# Autodesk Inventor assembly: LGA 771 Passive Heatsink
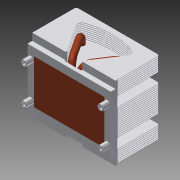
[picture p0: Inventor's stored thumbnail of the model, 180x180]
Saved by Autodesk Inventor 2015 (Build 190159000, 159)
## iProperties
Created: 2015-08-21
Part Number: LGA 771 Passive Heatsink
Document SubType Name: Assembly
Designer: Kyle
Author: Kyle
## Documents named in this file (7)
- C:\Users\Kyle\Documents\Project documentation\Supermicro X7DCA-L Watercooling\LGA 771 Passive Heatsink.iam
- C:\Users\Kyle\Documents\Project documentation\Supermicro X7DCA-L Watercooling\Heatsink_base_al.ipt
- C:\Users\Kyle\Documents\Project documentation\Supermicro X7DCA-L Watercooling\Heatsink_base_cu.ipt
- C:\Users\Kyle\Documents\Project documentation\Supermicro X7DCA-L Watercooling\Fin_full.ipt
- C:\Users\Kyle\Documents\Project documentation\Supermicro X7DCA-L Watercooling\Fin_short.ipt
- C:\Users\Kyle\Documents\Project documentation\Supermicro X7DCA-L Watercooling\Fin_holed.ipt
- C:\Users\Kyle\Documents\Project documentation\Supermicro X7DCA-L Watercooling\Heatpipe.iam
## Components (47 placed, 6 different names)
1. Heatsink_base_al:1 — Mate:1, Mate:2, Flush:1, Mate:7, Flush:2, Flush:3, Mate:8, Flush:4, Mate:10, Flush:5, Mate:12, Flush:6, Mate:14, Flush:7, Mate:16, Flush:8, Mate:18, Flush:9, Mate:20, Flush:10, Mate:22, Flush:11, Mate:24, Mate:26, Mate:28, Mate:30, Mate:32, Flush:16, Mate:34, Flush:17, Mate:36, Flush:18, Mate:38, Flush:19, Mate:40, Flush:20, Mate:42, Flush:21, Mate:44, Flush:22, Mate:46, Flush:23, Mate:48, Flush:24, Mate:50, Flush:25, Mate:52, Flush:26, Mate:54, Flush:27, Mate:56, Flush:28, Mate:58, Flush:29, Mate:60, Flush:30, Mate:62, Flush:31, Mate:64, Mate:66, Mate:68, Mate:70, Mate:72, Mate:74, Flush:37, Mate:76, Flush:38, Mate:78, Flush:39, Mate:80, Flush:40, Mate:82, Flush:41, Mate:84, Flush:42, Mate:86, Flush:43, Mate:88, Flush:44, Mate:90, Flush:45
2. Heatsink_base_cu:1 — Mate:1, Mate:2, Flush:1, Mate:92, Mate:93, Mate:94, Mate:95
3. Fin_full:1 — Mate:7, Flush:2, Flush:3, Mate:9, Tangent:1, Tangent:2, Tangent:3
4. Fin_full:2 — Mate:20, Flush:10, Mate:21, Mate:23
5. Fin_full:3 — Mate:18, Flush:9, Mate:19, Mate:21
6. Fin_full:4 — Mate:16, Flush:8, Mate:17, Mate:19
7. Fin_full:5 — Mate:12, Flush:6, Mate:13, Mate:15
8. Fin_full:6 — Mate:10, Flush:5, Mate:11, Mate:13
9. Fin_full:7 — Mate:8, Flush:4, Mate:9, Mate:11
10. Fin_full:8 — Mate:14, Flush:7, Mate:15, Mate:17
11. Fin_short:1 — Mate:30, Flush:15, Mate:31, Mate:33, Flush:32
12. Fin_short:2 — Mate:28, Mate:29, Flush:14, Flush:15, Mate:31
13. Fin_short:3 — Mate:26, Flush:13, Mate:27, Mate:29, Flush:14
14. Fin_short:4 — Mate:24, Flush:12, Mate:25, Flush:13, Mate:27
15. Fin_short:5 — Mate:22, Flush:11, Mate:23, Flush:12, Mate:25
16. Fin_full:9 — Mate:62, Flush:31, Mate:63, Mate:65
17. Fin_full:10 — Mate:60, Flush:30, Mate:61, Mate:63
18. Fin_full:11 — Mate:58, Flush:29, Mate:59, Mate:61
19. Fin_full:12 — Mate:56, Flush:28, Mate:57, Mate:59
20. Fin_full:13 — Mate:54, Flush:27, Mate:55, Mate:57
21. Fin_full:14 — Mate:52, Flush:26, Mate:53, Mate:55
22. Fin_full:15 — Mate:50, Flush:25, Mate:51, Mate:53
23. Fin_full:16 — Mate:48, Flush:24, Mate:49, Mate:51
24. Fin_full:17 — Mate:46, Flush:23, Mate:47, Mate:49
25. Fin_full:18 — Mate:44, Flush:22, Mate:45, Mate:47
26. Fin_full:19 — Mate:42, Flush:21, Mate:43, Mate:45
27. Fin_full:20 — Mate:40, Flush:20, Mate:41, Mate:43
28. Fin_full:21 — Mate:38, Flush:19, Mate:39, Mate:41
29. Fin_full:22 — Mate:36, Flush:18, Mate:37, Mate:39
30. Fin_full:23 — Mate:34, Flush:17, Mate:35, Mate:37
31. Fin_full:24 — Mate:32, Flush:16, Mate:33, Mate:35
32. Fin_short:6 — Mate:72, Flush:36, Mate:73, Mate:75
33. Fin_short:7 — Mate:70, Flush:35, Mate:71, Flush:36, Mate:73
34. Fin_short:8 — Mate:68, Flush:34, Mate:69, Flush:35, Mate:71
35. Fin_short:9 — Mate:66, Flush:33, Mate:67, Flush:34, Mate:69
36. Fin_short:10 — Mate:64, Flush:32, Mate:65, Flush:33, Mate:67
37. Fin_holed:1 — Mate:90, Flush:45, Mate:91
38. Fin_holed:2 — Mate:88, Flush:44, Mate:89, Mate:91
39. Fin_holed:3 — Mate:86, Flush:43, Mate:87, Mate:89
40. Fin_holed:4 — Mate:84, Flush:42, Mate:85, Mate:87
41. Fin_holed:5 — Mate:76, Flush:38, Mate:77, Mate:79
42. Fin_holed:6 — Mate:82, Flush:41, Mate:83, Mate:85
43. Fin_holed:7 — Mate:80, Flush:40, Mate:81, Mate:83
44. Fin_holed:8 — Mate:78, Flush:39, Mate:79, Mate:81
45. Fin_holed:9 — Mate:74, Flush:37, Mate:75, Mate:77
46. Heatpipe:1 [sub-assembly] — Mate:92, Mate:95, Tangent:3
47. Heatpipe:2 [sub-assembly] — Mate:93, Mate:94, Tangent:1, Tangent:2
## Relationships (139: Mate 91, Flush 45, Tangent 3)
- Mate:1: Heatsink_base_al:1 ↔ Heatsink_base_cu:1
- Mate:2: Heatsink_base_al:1 ↔ Heatsink_base_cu:1
- Flush:1: Heatsink_base_al:1 ↔ Heatsink_base_cu:1
- Mate:7: Heatsink_base_al:1 ↔ Fin_full:1
- Flush:2: Heatsink_base_al:1 ↔ Fin_full:1
- Flush:3: Heatsink_base_al:1 ↔ Fin_full:1
- Mate:8: Heatsink_base_al:1 ↔ Fin_full:7
- Flush:4: Heatsink_base_al:1 ↔ Fin_full:7
- Mate:9: Fin_full:1 ↔ Fin_full:7
- Mate:10: Heatsink_base_al:1 ↔ Fin_full:6
- Flush:5: Heatsink_base_al:1 ↔ Fin_full:6
- Mate:11: Fin_full:6 ↔ Fin_full:7
- Mate:12: Heatsink_base_al:1 ↔ Fin_full:5
- Flush:6: Heatsink_base_al:1 ↔ Fin_full:5
- Mate:13: Fin_full:5 ↔ Fin_full:6
- Mate:14: Heatsink_base_al:1 ↔ Fin_full:8
- Flush:7: Heatsink_base_al:1 ↔ Fin_full:8
- Mate:15: Fin_full:5 ↔ Fin_full:8
- Mate:16: Heatsink_base_al:1 ↔ Fin_full:4
- Flush:8: Heatsink_base_al:1 ↔ Fin_full:4
- Mate:17: Fin_full:4 ↔ Fin_full:8
- Mate:18: Heatsink_base_al:1 ↔ Fin_full:3
- Flush:9: Heatsink_base_al:1 ↔ Fin_full:3
- Mate:19: Fin_full:3 ↔ Fin_full:4
- Mate:20: Heatsink_base_al:1 ↔ Fin_full:2
- Flush:10: Heatsink_base_al:1 ↔ Fin_full:2
- Mate:21: Fin_full:2 ↔ Fin_full:3
- Mate:22: Heatsink_base_al:1 ↔ Fin_short:5
- Flush:11 (10.16 mm): Heatsink_base_al:1 ↔ Fin_short:5
- Mate:23: Fin_full:2 ↔ Fin_short:5
- Mate:24: Heatsink_base_al:1 ↔ Fin_short:4
- Flush:12: Fin_short:4 ↔ Fin_short:5
- Mate:25: Fin_short:4 ↔ Fin_short:5
- Mate:26: Heatsink_base_al:1 ↔ Fin_short:3
- Flush:13: Fin_short:3 ↔ Fin_short:4
- Mate:27: Fin_short:3 ↔ Fin_short:4
- Mate:28: Heatsink_base_al:1 ↔ Fin_short:2
- Mate:29: Fin_short:2 ↔ Fin_short:3
- Flush:14: Fin_short:2 ↔ Fin_short:3
- Mate:30: Heatsink_base_al:1 ↔ Fin_short:1
- Flush:15: Fin_short:1 ↔ Fin_short:2
- Mate:31: Fin_short:1 ↔ Fin_short:2
- Mate:32: Heatsink_base_al:1 ↔ Fin_full:24
- Flush:16: Heatsink_base_al:1 ↔ Fin_full:24
- Mate:33: Fin_short:1 ↔ Fin_full:24
- Mate:34: Heatsink_base_al:1 ↔ Fin_full:23
- Flush:17: Heatsink_base_al:1 ↔ Fin_full:23
- Mate:35: Fin_full:23 ↔ Fin_full:24
- Mate:36: Heatsink_base_al:1 ↔ Fin_full:22
- Flush:18: Heatsink_base_al:1 ↔ Fin_full:22
- Mate:37: Fin_full:22 ↔ Fin_full:23
- Mate:38: Heatsink_base_al:1 ↔ Fin_full:21
- Flush:19: Heatsink_base_al:1 ↔ Fin_full:21
- Mate:39: Fin_full:21 ↔ Fin_full:22
- Mate:40: Heatsink_base_al:1 ↔ Fin_full:20
- Flush:20: Heatsink_base_al:1 ↔ Fin_full:20
- Mate:41: Fin_full:20 ↔ Fin_full:21
- Mate:42: Heatsink_base_al:1 ↔ Fin_full:19
- Flush:21: Heatsink_base_al:1 ↔ Fin_full:19
- Mate:43: Fin_full:19 ↔ Fin_full:20
- Mate:44: Heatsink_base_al:1 ↔ Fin_full:18
- Flush:22: Heatsink_base_al:1 ↔ Fin_full:18
- Mate:45: Fin_full:18 ↔ Fin_full:19
- Mate:46: Heatsink_base_al:1 ↔ Fin_full:17
- Flush:23: Heatsink_base_al:1 ↔ Fin_full:17
- Mate:47: Fin_full:17 ↔ Fin_full:18
- Mate:48: Heatsink_base_al:1 ↔ Fin_full:16
- Flush:24: Heatsink_base_al:1 ↔ Fin_full:16
- Mate:49: Fin_full:16 ↔ Fin_full:17
- Mate:50: Heatsink_base_al:1 ↔ Fin_full:15
- Flush:25: Heatsink_base_al:1 ↔ Fin_full:15
- Mate:51: Fin_full:15 ↔ Fin_full:16
- Mate:52: Heatsink_base_al:1 ↔ Fin_full:14
- Flush:26: Heatsink_base_al:1 ↔ Fin_full:14
- Mate:53: Fin_full:14 ↔ Fin_full:15
- Mate:54: Heatsink_base_al:1 ↔ Fin_full:13
- Flush:27: Heatsink_base_al:1 ↔ Fin_full:13
- Mate:55: Fin_full:13 ↔ Fin_full:14
- Mate:56: Heatsink_base_al:1 ↔ Fin_full:12
- Flush:28: Heatsink_base_al:1 ↔ Fin_full:12
- Mate:57: Fin_full:12 ↔ Fin_full:13
- Mate:58: Heatsink_base_al:1 ↔ Fin_full:11
- Flush:29: Heatsink_base_al:1 ↔ Fin_full:11
- Mate:59: Fin_full:11 ↔ Fin_full:12
- Mate:60: Heatsink_base_al:1 ↔ Fin_full:10
- Flush:30: Heatsink_base_al:1 ↔ Fin_full:10
- Mate:61: Fin_full:10 ↔ Fin_full:11
- Mate:62: Heatsink_base_al:1 ↔ Fin_full:9
- Flush:31: Heatsink_base_al:1 ↔ Fin_full:9
- Mate:63: Fin_full:9 ↔ Fin_full:10
- Mate:64: Heatsink_base_al:1 ↔ Fin_short:10
- Flush:32: Fin_short:1 ↔ Fin_short:10
- Mate:65: Fin_full:9 ↔ Fin_short:10
- Mate:66: Heatsink_base_al:1 ↔ Fin_short:9
- Flush:33: Fin_short:9 ↔ Fin_short:10
- Mate:67: Fin_short:9 ↔ Fin_short:10
- Mate:68: Heatsink_base_al:1 ↔ Fin_short:8
- Flush:34: Fin_short:8 ↔ Fin_short:9
- Mate:69: Fin_short:8 ↔ Fin_short:9
- Mate:70: Heatsink_base_al:1 ↔ Fin_short:7
- Flush:35: Fin_short:7 ↔ Fin_short:8
- Mate:71: Fin_short:7 ↔ Fin_short:8
- Mate:72: Heatsink_base_al:1 ↔ Fin_short:6
- Flush:36: Fin_short:6 ↔ Fin_short:7
- Mate:73: Fin_short:6 ↔ Fin_short:7
- Mate:74: Heatsink_base_al:1 ↔ Fin_holed:9
- Flush:37: Heatsink_base_al:1 ↔ Fin_holed:9
- Mate:75: Fin_short:6 ↔ Fin_holed:9
- Mate:76: Heatsink_base_al:1 ↔ Fin_holed:5
- Flush:38: Heatsink_base_al:1 ↔ Fin_holed:5
- Mate:77: Fin_holed:5 ↔ Fin_holed:9
- Mate:78: Heatsink_base_al:1 ↔ Fin_holed:8
- Flush:39: Heatsink_base_al:1 ↔ Fin_holed:8
- Mate:79: Fin_holed:5 ↔ Fin_holed:8
- Mate:80: Heatsink_base_al:1 ↔ Fin_holed:7
- Flush:40: Heatsink_base_al:1 ↔ Fin_holed:7
- Mate:81: Fin_holed:7 ↔ Fin_holed:8
- Mate:82: Heatsink_base_al:1 ↔ Fin_holed:6
- Flush:41: Heatsink_base_al:1 ↔ Fin_holed:6
- Mate:83: Fin_holed:6 ↔ Fin_holed:7
- Mate:84: Heatsink_base_al:1 ↔ Fin_holed:4
- Flush:42: Heatsink_base_al:1 ↔ Fin_holed:4
- Mate:85: Fin_holed:4 ↔ Fin_holed:6
- Mate:86: Heatsink_base_al:1 ↔ Fin_holed:3
- Flush:43: Heatsink_base_al:1 ↔ Fin_holed:3
- Mate:87: Fin_holed:3 ↔ Fin_holed:4
- Mate:88: Heatsink_base_al:1 ↔ Fin_holed:2
- Flush:44: Heatsink_base_al:1 ↔ Fin_holed:2
- Mate:89: Fin_holed:2 ↔ Fin_holed:3
- Mate:90: Heatsink_base_al:1 ↔ Fin_holed:1
- Flush:45: Heatsink_base_al:1 ↔ Fin_holed:1
- Mate:91: Fin_holed:1 ↔ Fin_holed:2
- Mate:92: Heatsink_base_cu:1 ↔ Heatpipe:1
- Mate:93: Heatsink_base_cu:1 ↔ Heatpipe:2
- Mate:94: Heatsink_base_cu:1 ↔ Heatpipe:2
- Mate:95: Heatsink_base_cu:1 ↔ Heatpipe:1
- Tangent:1: Fin_full:1 ↔ Heatpipe:2
- Tangent:2: Fin_full:1 ↔ Heatpipe:2
- Tangent:3: Fin_full:1 ↔ Heatpipe:1
